# Autodesk Inventor assembly: 5_left_Arm_joint
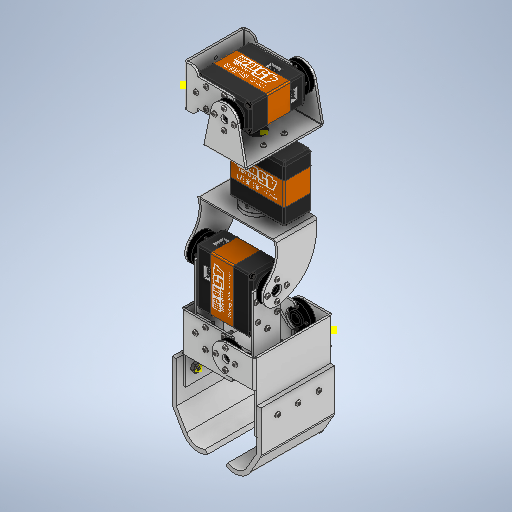
[picture p0: Inventor's stored thumbnail of the model, 512x512]
Saved by Autodesk Inventor 2026.1 (Build 301233020, 233B)
## iProperties
Created: 2026-01-04
Part Number: 5_left_Arm_joint
Document SubType Name: Assembly
Designer: aa992
Author: aa992
## Documents named in this file (18)
- C:\Users\aa992\OneDrive\Desktop\RHp_Humanoid_ver1\Assembly\5_left_Arm_joint.iam
- C:\Users\aa992\OneDrive\Desktop\RHp_Humanoid_ver1\Part\Frame\Arm\axis_13_top_frame.ipt
- C:\Users\aa992\OneDrive\Desktop\RHp_Humanoid_ver1\Part\HTD-45H, Horn\HTD-45H\HTD-45H.iam
- C:\Users\aa992\OneDrive\Desktop\RHp_Humanoid_ver1\Part\HTD-45H, Horn\Horn\Top Horn.ipt
- C:\Users\aa992\OneDrive\Desktop\RHp_Humanoid_ver1\Part\HTD-45H, Horn\Horn\Bottom Horn.ipt
- C:\Users\aa992\OneDrive\Desktop\RHp_Humanoid_ver1\Part\Frame\Arm\axis_14_bottom_frame.ipt
- C:\Users\aa992\OneDrive\Desktop\RHp_Humanoid_ver1\Part\HTD-45H, Horn\Horn\Top Horn silver.ipt
- C:\Users\aa992\OneDrive\Desktop\RHp_Humanoid_ver1\Part\Frame\Arm\axis_15_bottom_frame.ipt
- C:\Users\aa992\OneDrive\Desktop\RHp_Humanoid_ver1\Part\Frame\Arm\axis_16_top_frame.ipt
- C:\Users\aa992\OneDrive\Desktop\RHp_Humanoid_ver1\Part\Frame\Arm\axis_16_bottom_frame.ipt
- C:\Users\aa992\OneDrive\Desktop\RHp_Humanoid_ver1\Part\Frame\Arm\axis_17_top_frame.ipt
- C:\Users\aa992\OneDrive\Desktop\RHp_Humanoid_ver1\Part\Frame\Arm\axis_17_bottom_frame.ipt
- C:\Users\aa992\OneDrive\Desktop\RHp_Humanoid_ver1\Part\Frame\Arm\gripper_frame.ipt
- C:\Users\aa992\OneDrive\Desktop\RHp_Humanoid_ver1\Part\Bolt, Bearing, Nut, Washer\M2x6 Round Bolt.ipt
- C:\Users\aa992\OneDrive\Desktop\RHp_Humanoid_ver1\Part\Bolt, Bearing, Nut, Washer\볼트, 너트\M3x8 Bolt.ipt
- C:\Users\aa992\OneDrive\Desktop\RHp_Humanoid_ver1\Part\Bolt, Bearing, Nut, Washer\볼트, 너트\M3 Nut.ipt
- C:\Users\aa992\OneDrive\Desktop\RHp_Humanoid_ver1\Part\Bolt, Bearing, Nut, Washer\볼트, 너트\M2x8 Bolt.ipt
- C:\Users\aa992\OneDrive\Desktop\RHp_Humanoid_ver1\Part\Bolt, Bearing, Nut, Washer\볼트, 너트\M2x4 Bolt.ipt
## Components (99 placed, 17 different names)
1. axis_13_top_frame:1 — Mate:1, Flush:1, Flush:2, Rigid:1, Rigid:19, Rigid:20, Rigid:21, Rigid:22, Rigid:23, Rigid:24, Rigid:25, Rigid:26, Rigid:27
2. HTD-45H:1 [sub-assembly] — Rigid:1, Rotational:1, Rigid:2
3. Top Horn:1 — Rotational:1
4. Bottom Horn:1 — Rigid:2, Rigid:18
5. axis_14_bottom_frame:1 — Rigid:4, Rigid:18, Rigid:28, Rigid:29, Rigid:30, Rigid:31, Rigid:32, Rigid:33, Rigid:34, Rigid:35, Rigid:94, Rigid:95, Rigid:96, Rigid:97
6. HTD-45H:2 [sub-assembly] — Rigid:4, Rotational:2
7. Top Horn silver:1 — Rotational:2, Rigid:5
8. axis_15_bottom_frame:1 — Rigid:5, Rigid:9, Rigid:10, Rigid:36, Rigid:37, Rigid:38, Rigid:39, Rigid:40, Rigid:41, Rigid:42, Rigid:43, Rigid:44, Rigid:45, Rigid:46, Rigid:47
9. Top Horn:2 — Rotational:3, Rigid:10
10. Bottom Horn:2 — Rigid:9
11. HTD-45H:3 [sub-assembly] — Rotational:3, Rigid:8
12. axis_16_top_frame:1 — Rigid:8, Rigid:11, Rigid:48, Rigid:49, Rigid:50, Rigid:51, Rigid:52, Rigid:53, Rigid:54, Rigid:55, Rigid:56, Rigid:74, Rigid:75, Rigid:76, Rigid:77
13. axis_16_bottom_frame:1 — Rigid:11, Rigid:12, Rigid:14, Rigid:78, Rigid:79, Rigid:80, Rigid:81
14. HTD-45H:4 [sub-assembly] — Rigid:12, Rotational:4, Rigid:13
15. Top Horn:3 — Rotational:4, Rigid:15
16. Bottom Horn:3 — Rigid:13
17. axis_17_top_frame:1 — Rigid:14, Rigid:16, Rigid:65, Rigid:66, Rigid:67, Rigid:68, Rigid:69, Rigid:70, Rigid:71, Rigid:72, Rigid:73, Rigid:88, Rigid:89, Rigid:90
18. axis_17_bottom_frame:1 — Rigid:15, Rigid:17, Rigid:57, Rigid:58, Rigid:59, Rigid:60, Rigid:61, Rigid:62, Rigid:63, Rigid:64, Rigid:91, Rigid:92, Rigid:93
19. gripper_frame:1 — Rigid:16, Rigid:82, Rigid:83, Rigid:84
20. gripper_frame:2 — Rigid:17, Rigid:85, Rigid:86, Rigid:87
21. M2x6 Round Bolt:1 — Rigid:21
22. M2x6 Round Bolt:2 — Rigid:20
23. M2x6 Round Bolt:3 — Rigid:19
24. M2x6 Round Bolt:4 — Rigid:23
25. M2x6 Round Bolt:5 — Rigid:22
26. M2x6 Round Bolt:6 — Rigid:24
27. M2x6 Round Bolt:7 — Rigid:25
28. M2x6 Round Bolt:8 — Rigid:27
29. M2x6 Round Bolt:9 — Rigid:26
30. M2x6 Round Bolt:10 — Rigid:30
31. M2x6 Round Bolt:11 — Rigid:28
32. M2x6 Round Bolt:12 — Rigid:31
33. M2x6 Round Bolt:13 — Rigid:29
34. M2x6 Round Bolt:14 — Rigid:32
35. M2x6 Round Bolt:15 — Rigid:33
36. M2x6 Round Bolt:16 — Rigid:34
37. M2x6 Round Bolt:17 — Rigid:35
38. M2x6 Round Bolt:22 — Rigid:38
39. M2x6 Round Bolt:23 — Rigid:36
40. M2x6 Round Bolt:24 — Rigid:39
41. M2x6 Round Bolt:25 — Rigid:37
42. M2x6 Round Bolt:26 — Rigid:42
43. M2x6 Round Bolt:27 — Rigid:40
44. M2x6 Round Bolt:28 — Rigid:43
45. M2x6 Round Bolt:29 — Rigid:41
46. M2x6 Round Bolt:30 — Rigid:44
47. M2x6 Round Bolt:31 — Rigid:45
48. M2x6 Round Bolt:32 — Rigid:47
49. M2x6 Round Bolt:33 — Rigid:46
50. M2x6 Round Bolt:34 — Rigid:48
51. M2x6 Round Bolt:35 — Rigid:49
52. M2x6 Round Bolt:36 — Rigid:51
53. M2x6 Round Bolt:37 — Rigid:50
54. M2x6 Round Bolt:38 — Rigid:55
55. M2x6 Round Bolt:39 — Rigid:53
56. M2x6 Round Bolt:40 — Rigid:54
57. M2x6 Round Bolt:41 — Rigid:52
58. M2x6 Round Bolt:42 — Rigid:56
59. M2x6 Round Bolt:43 — Rigid:58
60. M2x6 Round Bolt:44 — Rigid:57
61. M2x6 Round Bolt:45 — Rigid:60
62. M2x6 Round Bolt:46 — Rigid:59
63. M2x6 Round Bolt:47 — Rigid:61
64. M2x6 Round Bolt:48 — Rigid:62
65. M2x6 Round Bolt:49 — Rigid:64
66. M2x6 Round Bolt:50 — Rigid:63
67. M2x6 Round Bolt:51 — Rigid:66
68. M2x6 Round Bolt:52 — Rigid:69
69. M2x6 Round Bolt:53 — Rigid:67
70. M2x6 Round Bolt:54 — Rigid:68
71. M2x6 Round Bolt:55 — Rigid:65
72. M2x6 Round Bolt:56 — Rigid:71
73. M2x6 Round Bolt:57 — Rigid:72
74. M2x6 Round Bolt:58 — Rigid:70
75. M2x6 Round Bolt:59 — Rigid:73
76. M3x8 Bolt:1 — Rigid:74
77. M3x8 Bolt:2 — Rigid:76
78. M3x8 Bolt:3 — Rigid:75
79. M3x8 Bolt:4 — Rigid:77
80. M3 Nut:1 — Rigid:78
81. M3 Nut:2 — Rigid:80
82. M3 Nut:3 — Rigid:79
83. M3 Nut:4 — Rigid:81
84. M2x8 Bolt:1 — Rigid:82
85. M2x8 Bolt:2 — Rigid:84
86. M2x8 Bolt:3 — Rigid:83
87. M2x8 Bolt:4 — Rigid:85
88. M2x8 Bolt:5 — Rigid:86
89. M2x8 Bolt:6 — Rigid:87
90. M3 Nut:5 — Rigid:88
91. M3 Nut:6 — Rigid:89
92. M3 Nut:7 — Rigid:90
93. M3 Nut:8 — Rigid:92
94. M3 Nut:9 — Rigid:93
95. M3 Nut:10 — Rigid:91
96. M2x4 Bolt:1 — Rigid:94
97. M2x4 Bolt:2 — Rigid:95
98. M2x4 Bolt:3 — Rigid:96
99. M2x4 Bolt:4 — Rigid:97
## Relationships (101: WeldJoint 94, RevoluteJoint 4, Flush 2, Mate 1)
- Mate:1: axis_13_top_frame:1
- Flush:1: axis_13_top_frame:1
- Flush:2: axis_13_top_frame:1
- Rigid:1 [WeldJoint]: axis_13_top_frame:1 ↔ HTD-45H:1
- Rotational:1 [RevoluteJoint]: HTD-45H:1 ↔ Top Horn:1
- Rigid:2 [WeldJoint]: HTD-45H:1 ↔ Bottom Horn:1
- Rigid:4 [WeldJoint]: axis_14_bottom_frame:1 ↔ HTD-45H:2
- Rotational:2 [RevoluteJoint]: HTD-45H:2 ↔ Top Horn silver:1
- Rigid:5 [WeldJoint]: Top Horn silver:1 ↔ axis_15_bottom_frame:1
- Rotational:3 [RevoluteJoint]: Top Horn:2 ↔ HTD-45H:3
- Rigid:8 [WeldJoint]: HTD-45H:3 ↔ axis_16_top_frame:1
- Rigid:9 [WeldJoint]: axis_15_bottom_frame:1 ↔ Bottom Horn:2
- Rigid:10 [WeldJoint]: axis_15_bottom_frame:1 ↔ Top Horn:2
- Rigid:11 [WeldJoint]: axis_16_top_frame:1 ↔ axis_16_bottom_frame:1
- Rigid:12 [WeldJoint]: axis_16_bottom_frame:1 ↔ HTD-45H:4
- Rotational:4 [RevoluteJoint]: HTD-45H:4 ↔ Top Horn:3
- Rigid:13 [WeldJoint]: HTD-45H:4 ↔ Bottom Horn:3
- Rigid:14 [WeldJoint]: axis_16_bottom_frame:1 ↔ axis_17_top_frame:1
- Rigid:15 [WeldJoint]: Top Horn:3 ↔ axis_17_bottom_frame:1
- Rigid:16 [WeldJoint]: axis_17_top_frame:1 ↔ gripper_frame:1
- Rigid:17 [WeldJoint]: axis_17_bottom_frame:1 ↔ gripper_frame:2
- Rigid:18 [WeldJoint]: Bottom Horn:1 ↔ axis_14_bottom_frame:1
- Rigid:19 [WeldJoint]: axis_13_top_frame:1 ↔ M2x6 Round Bolt:3
- Rigid:20 [WeldJoint]: axis_13_top_frame:1 ↔ M2x6 Round Bolt:2
- Rigid:21 [WeldJoint]: axis_13_top_frame:1 ↔ M2x6 Round Bolt:1
- Rigid:22 [WeldJoint]: axis_13_top_frame:1 ↔ M2x6 Round Bolt:5
- Rigid:23 [WeldJoint]: axis_13_top_frame:1 ↔ M2x6 Round Bolt:4
- Rigid:24 [WeldJoint]: axis_13_top_frame:1 ↔ M2x6 Round Bolt:6
- Rigid:25 [WeldJoint]: axis_13_top_frame:1 ↔ M2x6 Round Bolt:7
- Rigid:26 [WeldJoint]: axis_13_top_frame:1 ↔ M2x6 Round Bolt:9
- Rigid:27 [WeldJoint]: axis_13_top_frame:1 ↔ M2x6 Round Bolt:8
- Rigid:28 [WeldJoint]: axis_14_bottom_frame:1 ↔ M2x6 Round Bolt:11
- Rigid:29 [WeldJoint]: axis_14_bottom_frame:1 ↔ M2x6 Round Bolt:13
- Rigid:30 [WeldJoint]: axis_14_bottom_frame:1 ↔ M2x6 Round Bolt:10
- Rigid:31 [WeldJoint]: axis_14_bottom_frame:1 ↔ M2x6 Round Bolt:12
- Rigid:32 [WeldJoint]: axis_14_bottom_frame:1 ↔ M2x6 Round Bolt:14
- Rigid:33 [WeldJoint]: axis_14_bottom_frame:1 ↔ M2x6 Round Bolt:15
- Rigid:34 [WeldJoint]: axis_14_bottom_frame:1 ↔ M2x6 Round Bolt:16
- Rigid:35 [WeldJoint]: axis_14_bottom_frame:1 ↔ M2x6 Round Bolt:17
- Rigid:36 [WeldJoint]: axis_15_bottom_frame:1 ↔ M2x6 Round Bolt:23
- Rigid:37 [WeldJoint]: axis_15_bottom_frame:1 ↔ M2x6 Round Bolt:25
- Rigid:38 [WeldJoint]: axis_15_bottom_frame:1 ↔ M2x6 Round Bolt:22
- Rigid:39 [WeldJoint]: axis_15_bottom_frame:1 ↔ M2x6 Round Bolt:24
- Rigid:40 [WeldJoint]: axis_15_bottom_frame:1 ↔ M2x6 Round Bolt:27
- Rigid:41 [WeldJoint]: axis_15_bottom_frame:1 ↔ M2x6 Round Bolt:29
- Rigid:42 [WeldJoint]: axis_15_bottom_frame:1 ↔ M2x6 Round Bolt:26
- Rigid:43 [WeldJoint]: axis_15_bottom_frame:1 ↔ M2x6 Round Bolt:28
- Rigid:44 [WeldJoint]: axis_15_bottom_frame:1 ↔ M2x6 Round Bolt:30
- Rigid:45 [WeldJoint]: axis_15_bottom_frame:1 ↔ M2x6 Round Bolt:31
- Rigid:46 [WeldJoint]: axis_15_bottom_frame:1 ↔ M2x6 Round Bolt:33
- Rigid:47 [WeldJoint]: axis_15_bottom_frame:1 ↔ M2x6 Round Bolt:32
- Rigid:48 [WeldJoint]: axis_16_top_frame:1 ↔ M2x6 Round Bolt:34
- Rigid:49 [WeldJoint]: axis_16_top_frame:1 ↔ M2x6 Round Bolt:35
- Rigid:50 [WeldJoint]: axis_16_top_frame:1 ↔ M2x6 Round Bolt:37
- Rigid:51 [WeldJoint]: axis_16_top_frame:1 ↔ M2x6 Round Bolt:36
- Rigid:52 [WeldJoint]: axis_16_top_frame:1 ↔ M2x6 Round Bolt:41
- Rigid:53 [WeldJoint]: axis_16_top_frame:1 ↔ M2x6 Round Bolt:39
- Rigid:54 [WeldJoint]: axis_16_top_frame:1 ↔ M2x6 Round Bolt:40
- Rigid:55 [WeldJoint]: axis_16_top_frame:1 ↔ M2x6 Round Bolt:38
- Rigid:56 [WeldJoint]: axis_16_top_frame:1 ↔ M2x6 Round Bolt:42
- Rigid:57 [WeldJoint]: axis_17_bottom_frame:1 ↔ M2x6 Round Bolt:44
- Rigid:58 [WeldJoint]: axis_17_bottom_frame:1 ↔ M2x6 Round Bolt:43
- Rigid:59 [WeldJoint]: axis_17_bottom_frame:1 ↔ M2x6 Round Bolt:46
- Rigid:60 [WeldJoint]: axis_17_bottom_frame:1 ↔ M2x6 Round Bolt:45
- Rigid:61 [WeldJoint]: axis_17_bottom_frame:1 ↔ M2x6 Round Bolt:47
- Rigid:62 [WeldJoint]: axis_17_bottom_frame:1 ↔ M2x6 Round Bolt:48
- Rigid:63 [WeldJoint]: axis_17_bottom_frame:1 ↔ M2x6 Round Bolt:50
- Rigid:64 [WeldJoint]: axis_17_bottom_frame:1 ↔ M2x6 Round Bolt:49
- Rigid:65 [WeldJoint]: axis_17_top_frame:1 ↔ M2x6 Round Bolt:55
- Rigid:66 [WeldJoint]: axis_17_top_frame:1 ↔ M2x6 Round Bolt:51
- Rigid:67 [WeldJoint]: axis_17_top_frame:1 ↔ M2x6 Round Bolt:53
- Rigid:68 [WeldJoint]: axis_17_top_frame:1 ↔ M2x6 Round Bolt:54
- Rigid:69 [WeldJoint]: axis_17_top_frame:1 ↔ M2x6 Round Bolt:52
- Rigid:70 [WeldJoint]: axis_17_top_frame:1 ↔ M2x6 Round Bolt:58
- Rigid:71 [WeldJoint]: axis_17_top_frame:1 ↔ M2x6 Round Bolt:56
- Rigid:72 [WeldJoint]: axis_17_top_frame:1 ↔ M2x6 Round Bolt:57
- Rigid:73 [WeldJoint]: axis_17_top_frame:1 ↔ M2x6 Round Bolt:59
- Rigid:74 [WeldJoint]: axis_16_top_frame:1 ↔ M3x8 Bolt:1
- Rigid:75 [WeldJoint]: axis_16_top_frame:1 ↔ M3x8 Bolt:3
- Rigid:76 [WeldJoint]: axis_16_top_frame:1 ↔ M3x8 Bolt:2
- Rigid:77 [WeldJoint]: axis_16_top_frame:1 ↔ M3x8 Bolt:4
- Rigid:78 [WeldJoint]: axis_16_bottom_frame:1 ↔ M3 Nut:1
- Rigid:79 [WeldJoint]: axis_16_bottom_frame:1 ↔ M3 Nut:3
- Rigid:80 [WeldJoint]: axis_16_bottom_frame:1 ↔ M3 Nut:2
- Rigid:81 [WeldJoint]: axis_16_bottom_frame:1 ↔ M3 Nut:4
- Rigid:82 [WeldJoint]: gripper_frame:1 ↔ M2x8 Bolt:1
- Rigid:83 [WeldJoint]: gripper_frame:1 ↔ M2x8 Bolt:3
- Rigid:84 [WeldJoint]: gripper_frame:1 ↔ M2x8 Bolt:2
- Rigid:85 [WeldJoint]: gripper_frame:2 ↔ M2x8 Bolt:4
- Rigid:86 [WeldJoint]: gripper_frame:2 ↔ M2x8 Bolt:5
- Rigid:87 [WeldJoint]: gripper_frame:2 ↔ M2x8 Bolt:6
- Rigid:88 [WeldJoint]: axis_17_top_frame:1 ↔ M3 Nut:5
- Rigid:89 [WeldJoint]: axis_17_top_frame:1 ↔ M3 Nut:6
- Rigid:90 [WeldJoint]: axis_17_top_frame:1 ↔ M3 Nut:7
- Rigid:91 [WeldJoint]: axis_17_bottom_frame:1 ↔ M3 Nut:10
- Rigid:92 [WeldJoint]: axis_17_bottom_frame:1 ↔ M3 Nut:8
- Rigid:93 [WeldJoint]: axis_17_bottom_frame:1 ↔ M3 Nut:9
- Rigid:94 [WeldJoint]: axis_14_bottom_frame:1 ↔ M2x4 Bolt:1
- Rigid:95 [WeldJoint]: axis_14_bottom_frame:1 ↔ M2x4 Bolt:2
- Rigid:96 [WeldJoint]: axis_14_bottom_frame:1 ↔ M2x4 Bolt:3
- Rigid:97 [WeldJoint]: axis_14_bottom_frame:1 ↔ M2x4 Bolt:4
